# Autodesk Inventor assembly: 2026 Tiger Burn Head
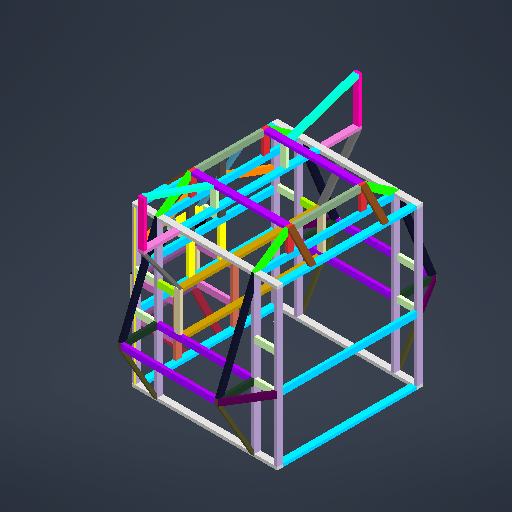
[picture p0: Inventor's stored thumbnail of the model, 512x512]
Saved by Autodesk Inventor 2027 (Build 310192000, 192)
## iProperties
Created: 2026-05-26
Part Number: 2026 Tiger Burn Head
Document SubType Name: Assembly
Designer: lucas
Author: lucas
## Documents named in this file (78)
- C:\Users\lucas\OneDrive\Documents\Inventor\Tiger Burn Head Frame 2026\2026 Tiger Burn Head.iam
- C:\Users\lucas\OneDrive\Documents\Inventor\Tiger Burn Head Frame 2026\2x4x96.ipt
- C:\Users\lucas\OneDrive\Documents\Inventor\Tiger Burn Head Frame 2026\2x4x88.ipt
- C:\Users\lucas\OneDrive\Documents\Inventor\Tiger Burn Head Frame 2026\2x4x101.ipt
- C:\Users\lucas\OneDrive\Documents\Inventor\Tiger Burn Head Frame 2026\2x4x24.ipt
- C:\Users\lucas\OneDrive\Documents\Inventor\Tiger Burn Head Frame 2026\2x4x26.ipt
- C:\Users\lucas\OneDrive\Documents\Inventor\Tiger Burn Head Frame 2026\2x4x39.ipt
- C:\Users\lucas\OneDrive\Documents\Inventor\Tiger Burn Head Frame 2026\2x4x38.ipt
- C:\Users\lucas\OneDrive\Documents\Inventor\Tiger Burn Head Frame 2026\Bottom jaw diagonals 2.ipt
- C:\Users\lucas\OneDrive\Documents\Inventor\Tiger Burn Head Frame 2026\Bottom jaw diagonals 2_MIR.ipt
- C:\Users\lucas\OneDrive\Documents\Inventor\Tiger Burn Head Frame 2026\2x4x24(with a cut).ipt
- C:\Users\lucas\OneDrive\Documents\Inventor\Tiger Burn Head Frame 2026\2x4x(24x43).ipt
- C:\Users\lucas\OneDrive\Documents\Inventor\Tiger Burn Head Frame 2026\Upper side diagonal.ipt
- C:\Users\lucas\OneDrive\Documents\Inventor\Tiger Burn Head Frame 2026\2x4x101_MIR.ipt
- C:\Users\lucas\OneDrive\Documents\Inventor\Tiger Burn Head Frame 2026\2x4x24(with a cut)_MIR.ipt
- C:\Users\lucas\OneDrive\Documents\Inventor\Tiger Burn Head Frame 2026\2x4x(24x43)_MIR.ipt
- C:\Users\lucas\OneDrive\Documents\Inventor\Tiger Burn Head Frame 2026\Upper side diagonal_MIR.ipt
- C:\Users\lucas\OneDrive\Documents\Inventor\Tiger Burn Head Frame 2026\2x4x101_MIR1.ipt
- C:\Users\lucas\OneDrive\Documents\Inventor\Tiger Burn Head Frame 2026\2x4x24(with a cut)_MIR1.ipt
- C:\Users\lucas\OneDrive\Documents\Inventor\Tiger Burn Head Frame 2026\2x4x(24x43)_MIR1.ipt
- C:\Users\lucas\OneDrive\Documents\Inventor\Tiger Burn Head Frame 2026\Upper side diagonal_MIR1.ipt
- C:\Users\lucas\OneDrive\Documents\Inventor\Tiger Burn Head Frame 2026\2x4x101_MIR_MIR.ipt
- C:\Users\lucas\OneDrive\Documents\Inventor\Tiger Burn Head Frame 2026\2x4x24(with a cut)_MIR_MIR.ipt
- C:\Users\lucas\OneDrive\Documents\Inventor\Tiger Burn Head Frame 2026\2x4x(24x43)_MIR_MIR.ipt
- C:\Users\lucas\OneDrive\Documents\Inventor\Tiger Burn Head Frame 2026\Upper side diagonal_MIR_MIR.ipt
- C:\Users\lucas\OneDrive\Documents\Inventor\Tiger Burn Head Frame 2026\Side piece.ipt
- C:\Users\lucas\OneDrive\Documents\Inventor\Tiger Burn Head Frame 2026\Side piece_MIR.ipt
- C:\Users\lucas\OneDrive\Documents\Inventor\Tiger Burn Head Frame 2026\2x4x15.ipt
- C:\Users\lucas\OneDrive\Documents\Inventor\Tiger Burn Head Frame 2026\2x4x44.ipt
- C:\Users\lucas\OneDrive\Documents\Inventor\Tiger Burn Head Frame 2026\Top of head diagonals.ipt
- C:\Users\lucas\OneDrive\Documents\Inventor\Tiger Burn Head Frame 2026\Top of head diagonals_MIR2.ipt
- C:\Users\lucas\OneDrive\Documents\Inventor\Tiger Burn Head Frame 2026\2x4x88_MIR.ipt
- C:\Users\lucas\OneDrive\Documents\Inventor\Tiger Burn Head Frame 2026\2x4x15_MIR1.ipt
- C:\Users\lucas\OneDrive\Documents\Inventor\Tiger Burn Head Frame 2026\2x4x44_MIR1.ipt
- C:\Users\lucas\OneDrive\Documents\Inventor\Tiger Burn Head Frame 2026\Top of head diagonals_MIR3.ipt
- C:\Users\lucas\OneDrive\Documents\Inventor\Tiger Burn Head Frame 2026\Top of head diagonals_MIR2_MIR.ipt
- C:\Users\lucas\OneDrive\Documents\Inventor\Tiger Burn Head Frame 2026\Side piece_MIR1.ipt
- C:\Users\lucas\OneDrive\Documents\Inventor\Tiger Burn Head Frame 2026\2x4x13.ipt
- C:\Users\lucas\OneDrive\Documents\Inventor\Tiger Burn Head Frame 2026\2x4x13_MIR.ipt
- C:\Users\lucas\OneDrive\Documents\Inventor\Tiger Burn Head Frame 2026\2x4x13_MIR1.ipt
- C:\Users\lucas\OneDrive\Documents\Inventor\Tiger Burn Head Frame 2026\2x4x13_MIR_MIR.ipt
- C:\Users\lucas\OneDrive\Documents\Inventor\Tiger Burn Head Frame 2026\2x4x88_MIR1.ipt
- C:\Users\lucas\OneDrive\Documents\Inventor\Tiger Burn Head Frame 2026\SideConnectors.ipt
- C:\Users\lucas\OneDrive\Documents\Inventor\Tiger Burn Head Frame 2026\SideConnectors_MIR.ipt
- C:\Users\lucas\OneDrive\Documents\Inventor\Tiger Burn Head Frame 2026\SideConnectors_MIR1.ipt
- C:\Users\lucas\OneDrive\Documents\Inventor\Tiger Burn Head Frame 2026\SideConnectors_MIR_MIR.ipt
- C:\Users\lucas\OneDrive\Documents\Inventor\Tiger Burn Head Frame 2026\Side piece_MIR2.ipt
- C:\Users\lucas\OneDrive\Documents\Inventor\Tiger Burn Head Frame 2026\Top Diagonals.ipt
- C:\Users\lucas\OneDrive\Documents\Inventor\Tiger Burn Head Frame 2026\Top Diagonals_MIR.ipt
- C:\Users\lucas\OneDrive\Documents\Inventor\Tiger Burn Head Frame 2026\Top Diagonals_MIR1.ipt
- C:\Users\lucas\OneDrive\Documents\Inventor\Tiger Burn Head Frame 2026\Top Diagonals_MIR_MIR.ipt
- C:\Users\lucas\OneDrive\Documents\Inventor\Tiger Burn Head Frame 2026\2x4x20.ipt
- C:\Users\lucas\OneDrive\Documents\Inventor\Tiger Burn Head Frame 2026\2x4x20_MIR.ipt
- C:\Users\lucas\OneDrive\Documents\Inventor\Tiger Burn Head Frame 2026\2x4x13_MIR2.ipt
- C:\Users\lucas\OneDrive\Documents\Inventor\Tiger Burn Head Frame 2026\Eyelids.ipt
- C:\Users\lucas\OneDrive\Documents\Inventor\Tiger Burn Head Frame 2026\Eyelids_MIR.ipt
- C:\Users\lucas\OneDrive\Documents\Inventor\Tiger Burn Head Frame 2026\UpperNoseDiagonalsv2.ipt
- C:\Users\lucas\OneDrive\Documents\Inventor\Tiger Burn Head Frame 2026\UpperNoseDiagonalsv2_MIR.ipt
- C:\Users\lucas\OneDrive\Documents\Inventor\Tiger Burn Head Frame 2026\Rename.ipt
- C:\Users\lucas\OneDrive\Documents\Inventor\Tiger Burn Head Frame 2026\Rename_MIR.ipt
- C:\Users\lucas\OneDrive\Documents\Inventor\Tiger Burn Head Frame 2026\Renamev2.ipt
- Eyelidpt2.ipt
- C:\Users\lucas\OneDrive\Documents\Inventor\Tiger Burn Head Frame 2026\Renamev2_MIR.ipt
- C:\Users\lucas\OneDrive\Documents\Inventor\Tiger Burn Head Frame 2026\LowerEarDiagonals.ipt
- C:\Users\lucas\OneDrive\Documents\Inventor\Tiger Burn Head Frame 2026\2x4x24_MIR1.ipt
- C:\Users\lucas\OneDrive\Documents\Inventor\Tiger Burn Head Frame 2026\2x4x26_MIR.ipt
- C:\Users\lucas\OneDrive\Documents\Inventor\Tiger Burn Head Frame 2026\LowerEarDiagonals_MIR.ipt
- C:\Users\lucas\OneDrive\Documents\Inventor\Tiger Burn Head Frame 2026\2x4x30.ipt
- C:\Users\lucas\OneDrive\Documents\Inventor\Tiger Burn Head Frame 2026\2x4x30_MIR.ipt
- C:\Users\lucas\OneDrive\Documents\Inventor\Tiger Burn Head Frame 2026\UpperEarDiagonalv2.ipt
- C:\Users\lucas\OneDrive\Documents\Inventor\Tiger Burn Head Frame 2026\UpperEarDiagonalv2_MIR.ipt
- C:\Users\lucas\OneDrive\Documents\Inventor\Tiger Burn Head Frame 2026\2x4x90.ipt
- C:\Users\lucas\OneDrive\Documents\Inventor\Tiger Burn Head Frame 2026\2x4x(Rename).ipt
- C:\Users\lucas\OneDrive\Documents\Inventor\Tiger Burn Head Frame 2026\2x4x13_MIR3.ipt
- C:\Users\lucas\OneDrive\Documents\Inventor\Tiger Burn Head Frame 2026\2x4x(Rename)_MIR.ipt
- C:\Users\lucas\OneDrive\Documents\Inventor\Tiger Burn Head Frame 2026\2x4x13_MIR4.ipt
- C:\Users\lucas\OneDrive\Documents\Inventor\Tiger Burn Head Frame 2026\2x4x13_MIR3_MIR.ipt
- C:\Users\lucas\OneDrive\Documents\Inventor\Tiger Burn Head Frame 2026\2x4x13_MIR5.ipt
## Components (107 placed, 77 different names)
1. 2x4x96:1 — Mate:1, Flush:1, Flush:2, Mate:2, Flush:3, Flush:4, Mate:8, Flush:15, Flush:16, Mate:9, Flush:17, Flush:18, Mate:28, Flush:53, Mate:38
2. 2x4x88:1 — Mate:1, Flush:1, Flush:2
3. 2x4x88:2 — Mate:2, Flush:3, Flush:4, Mate:3, Flush:5, Flush:6, Mate:12, Flush:23, Mate:13, Flush:25, Flush:52
4. 2x4x96:2 — Mate:3, Flush:5, Flush:6, Mate:7, Flush:13, Flush:14, Mate:10, Flush:19, Flush:20, Mate:39
5. 2x4x101:1 — Mate:7, Flush:13, Flush:14, Flush:24, Flush:107, Flush:108, Mate:68, Flush:123, Flush:136, Flush:137, Mate:73
6. 2x4x96:3 — Flush:21, Flush:22, Flush:87, Mate:72, Flush:139, Mate:78, Flush:149
7. 2x4x88:3
8. 2x4x88:4 — Flush:116, Flush:130
9. 2x4x96:4 — Mate:11, Mate:37
10. 2x4x101:2 — Mate:10, Flush:19, Flush:20, Mate:11, Flush:21, Flush:22
11. 2x4x101:3 — Mate:8, Flush:15, Flush:16, Flush:26, Flush:28, Flush:54, Mate:80, Flush:157
12. 2x4x101:4 — Mate:9, Flush:17, Flush:18
13. 2x4x39:1 — Mate:12, Flush:23, Flush:24, Mate:14
14. 2x4x39:2 — Mate:13, Flush:25, Flush:26, Flush:27, Flush:47
15. 2x4x88:5 — Mate:14, Flush:27, Flush:28, Mate:24, Flush:48, Mate:27, Flush:57, Mate:67, Flush:122
16. 2x4x24:1 — Mate:21, Flush:41, Flush:42
17. 2x4x24:2 — Mate:23, Flush:45, Flush:46, Mate:24, Flush:48
18. 2x4x24:3 — Mate:22, Flush:43, Flush:44
19. 2x4x24:4 — Mate:20, Flush:39, Flush:40
20. 2x4x26:2 — Mate:17, Flush:33, Flush:34, Mate:19, Flush:37, Flush:38, Mate:21, Flush:41, Flush:42, Mate:23, Flush:45, Flush:46, Flush:47, Flush:49, Flush:50
21. 2x4x38:2 — Mate:17, Flush:33, Flush:34, Mate:18, Flush:35, Flush:36, Mate:26
22. 2x4x26:3 — Mate:18, Flush:35, Flush:36, Mate:20, Flush:39, Flush:40, Mate:22, Flush:43, Flush:44, Flush:131, Flush:132
23. 2x4x38:3 — Mate:19, Flush:37, Flush:38, Mate:25
24. Bottom jaw diagonals 2:1 — Flush:49, Flush:50, Flush:52
25. Bottom jaw diagonals 2_MIR:1
26. 2x4x101:5 — Mate:28, Flush:53, Flush:54, Flush:56, Mate:30, Flush:95, Flush:105, Flush:106
27. 2x4x24(with a cut):1 — Flush:56, Mate:30, Flush:57, Flush:58, Flush:59, Flush:60, Flush:61, Flush:62
28. 2x4x(24x45) — Flush:58, Flush:59, Flush:72, Flush:73
29. Upper side diagonal:1 — Flush:60, Flush:61, Flush:62
30. 2x4x101_MIR:1 — Mate:31, Flush:63, Mate:53, Flush:88, Flush:94
31. 2x4x24(with a cut)_MIR:1 — Mate:31, Flush:63, Mate:32, Mate:33, Mate:34, Mate:35, Mate:36, Flush:76, Flush:109
32. 2x4x(24x43)_MIR:1 — Mate:32, Mate:33, Flush:75
33. Upper side diagonal_MIR:1 — Mate:34, Mate:35, Mate:36
34. 2x4x101_MIR1:1 — Mate:40, Flush:64, Mate:64, Flush:103
35. 2x4x24(with a cut)_MIR1:1 — Mate:40, Flush:64, Mate:41, Mate:42, Mate:43, Mate:44, Mate:45, Flush:74, Flush:104
36. 2x4x(24x43)_MIR1:1 — Mate:41, Mate:42
37. Upper side diagonal_MIR1:1 — Mate:43, Mate:44, Mate:45
38. 2x4x101_MIR_MIR:1 — Flush:65, Mate:46
39. 2x4x24(with a cut)_MIR_MIR:1 — Flush:65, Mate:46, Flush:66, Flush:67, Flush:68, Flush:69, Flush:70
40. 2x4x(24x43)_MIR_MIR:1 — Flush:66, Flush:67, Flush:71
41. Upper side diagonal_MIR_MIR:1 — Flush:68, Flush:69, Flush:70
42. 2x4x62 — Flush:71, Flush:72, Flush:73, Flush:74
43. Side piece_MIR:1 — Flush:75, Flush:76
44. 2x4x88:6 — Mate:53, Flush:87, Flush:88, Mate:55, Flush:93, Mate:56, Flush:96, Mate:57, Flush:97
45. 2x4x15:3 — Mate:55, Flush:93, Flush:94, Mate:66, Flush:114, Flush:115
46. 2x4x15:4 — Mate:56, Flush:95, Flush:96, Mate:58, Flush:161
47. 2x4x44:2
48. Top of head diagonals:2 — Mate:57, Flush:97, Mate:58
49. Top of head diagonals_MIR2:1
50. 2x4x88_MIR:1 — Flush:98, Mate:59, Flush:99, Mate:60, Flush:102, Mate:63, Flush:113
51. 2x4x15_MIR1:1 — Flush:98, Mate:59, Flush:100, Flush:101, Mate:61, Flush:110, Flush:111, Flush:112, Flush:113
52. 2x4x15_MIR1:2 — Flush:99, Mate:60, Mate:62
53. 2x4x44_MIR1:1 — Flush:100, Flush:101, Mate:61
54. Top of head diagonals_MIR3:1 — Mate:62, Flush:102, Mate:63
55. Top of head diagonals_MIR2_MIR:1 — Flush:112
56. Side piece:2 — Mate:64, Flush:103, Flush:104, Mate:79, Flush:156
57. Side piece_MIR1:1 — Mate:74, Flush:140
58. 2x4x13:1 — Flush:105, Flush:106
59. 2x4x13_MIR:1
60. 2x4x13_MIR1:1
61. 2x4x13_MIR_MIR:1
62. 2x4x88_MIR1:1 — Mate:65
63. SideConnectors:1 — Flush:107, Flush:108, Flush:109
64. SideConnectors_MIR:1
65. SideConnectors_MIR1:1
66. SideConnectors_MIR_MIR:1
67. Side piece:3 — Flush:110, Flush:111, Mate:66, Flush:152
68. Side piece_MIR2:1
69. Top Diagonals:1 — Flush:114, Flush:115, Flush:116
70. Top Diagonals_MIR:1
71. Top Diagonals_MIR1:1
72. Top Diagonals_MIR_MIR:1
73. 2x4x20:2 — Mate:67, Flush:122, Mate:69, Flush:124
74. 2x4x20_MIR:1
75. 2x4x88:7 — Mate:68, Flush:123, Mate:69, Flush:125, Mate:70, Flush:134, Flush:135, Flush:158
76. 2x4x13:2 — Flush:124, Flush:125, Mate:70, Flush:126, Mate:71, Flush:127, Flush:128, Flush:129, Flush:133
77. 2x4x13_MIR2:1
78. 2x4x20:3 — Flush:126, Mate:71, Flush:127
79. Eyelids:1 — Flush:128, Flush:129, Flush:130
80. Eyelids_MIR:1
81. UpperNoseDiagonalsv2:1 — Flush:131, Flush:132, Flush:133
82. UpperNoseDiagonalsv2_MIR:1
83. 2x4x34:1 — Flush:134, Flush:135, Flush:138
84. 2x4x34_MIR:1
85. Eyelidpt2:1 — Flush:136, Flush:137, Flush:138
86. Eyelidpt2_MIR:1
87. 2x4x24:5 — Mate:72, Flush:139, Mate:73, Flush:141, Flush:144, Flush:146, Flush:147, Flush:148
88. 2x4x26:4 — Mate:74, Flush:140, Flush:141, Flush:142, Flush:143, Flush:153, Flush:154
89. LowerEarDiagonals:1 — Flush:142, Flush:143, Flush:144
90. 2x4x24_MIR1:1 — Flush:145, Mate:75
91. 2x4x26_MIR:1 — Flush:145, Mate:76, Mate:77, Flush:155, Flush:159, Flush:160
92. LowerEarDiagonals_MIR:1 — Mate:75, Mate:76, Mate:77
93. 2x4x30:1 — Flush:146, Flush:147, Flush:150, Flush:151
94. 2x4x88:8 — Mate:78, Flush:148, Flush:149, Mate:81
95. 2x4x30_MIR:1
96. UpperEarDiagonalv2:1 — Flush:150, Flush:151, Flush:152
97. UpperEarDiagonalv2_MIR:1
98. 2x4x92:1 — Flush:153, Flush:154
99. 2x4x92:2 — Mate:79, Flush:155, Flush:156
100. 2x4x13:3 — Mate:80, Flush:157, Flush:158
101. 2x4x11:1 — Flush:159, Flush:160
102. 2x4x13_MIR3:1
103. 2x4x(Rename)_MIR:1
104. 2x4x13_MIR4:1
105. 2x4x13_MIR3_MIR:1
106. 2x4x13:4 — Mate:81, Flush:161
107. 2x4x13_MIR5:1
## Relationships (210: Flush 138, Mate 72)
- Mate:1: 2x4x96:1 ↔ 2x4x88:1
- Flush:1: 2x4x96:1 ↔ 2x4x88:1
- Flush:2: 2x4x96:1 ↔ 2x4x88:1
- Mate:2: 2x4x96:1 ↔ 2x4x88:2
- Flush:3: 2x4x96:1 ↔ 2x4x88:2
- Flush:4: 2x4x96:1 ↔ 2x4x88:2
- Mate:3: 2x4x88:2 ↔ 2x4x96:2
- Flush:5: 2x4x88:2 ↔ 2x4x96:2
- Flush:6: 2x4x88:2 ↔ 2x4x96:2
- [Mate]: 2x4x96:3 ↔ 2x4x88:3
- [Flush]: 2x4x96:3 ↔ 2x4x88:3
- [Flush]: 2x4x96:3 ↔ 2x4x88:3
- [Mate]: 2x4x96:3 ↔ 2x4x88:4
- [Flush]: 2x4x96:3 ↔ 2x4x88:4
- [Flush]: 2x4x96:3 ↔ 2x4x88:4
- [Mate]: 2x4x88:4 ↔ 2x4x96:4
- [Flush]: 2x4x88:4 ↔ 2x4x96:4
- [Flush]: 2x4x88:4 ↔ 2x4x96:4
- Mate:7: 2x4x96:2 ↔ 2x4x101:1
- Flush:13: 2x4x96:2 ↔ 2x4x101:1
- Flush:14: 2x4x96:2 ↔ 2x4x101:1
- Mate:8: 2x4x96:1 ↔ 2x4x101:3
- Flush:15: 2x4x96:1 ↔ 2x4x101:3
- Flush:16: 2x4x96:1 ↔ 2x4x101:3
- Mate:9: 2x4x96:1 ↔ 2x4x101:4
- Flush:17: 2x4x96:1 ↔ 2x4x101:4
- Flush:18: 2x4x96:1 ↔ 2x4x101:4
- Mate:10: 2x4x96:2 ↔ 2x4x101:2
- Flush:19: 2x4x96:2 ↔ 2x4x101:2
- Flush:20: 2x4x96:2 ↔ 2x4x101:2
- Mate:11: 2x4x96:4 ↔ 2x4x101:2
- Flush:21: 2x4x96:3 ↔ 2x4x101:2
- Flush:22: 2x4x96:3 ↔ 2x4x101:2
- Mate:12: 2x4x88:2 ↔ 2x4x39:1
- Flush:23: 2x4x88:2 ↔ 2x4x39:1
- Flush:24 (685.8 mm): 2x4x101:1 ↔ 2x4x39:1
- Mate:13: 2x4x88:2 ↔ 2x4x39:2
- Flush:25: 2x4x88:2 ↔ 2x4x39:2
- Flush:26 (685.8 mm): 2x4x101:3 ↔ 2x4x39:2
- Mate:14: 2x4x39:1 ↔ 2x4x88:5
- Flush:27: 2x4x39:2 ↔ 2x4x88:5
- Flush:28 (101.6 mm): 2x4x101:3 ↔ 2x4x88:5
- Mate:17: 2x4x26:2 ↔ 2x4x38:2
- Flush:33: 2x4x26:2 ↔ 2x4x38:2
- Flush:34: 2x4x26:2 ↔ 2x4x38:2
- Mate:18: 2x4x38:2 ↔ 2x4x26:3
- Flush:35: 2x4x38:2 ↔ 2x4x26:3
- Flush:36: 2x4x38:2 ↔ 2x4x26:3
- Mate:19: 2x4x26:2 ↔ 2x4x38:3
- Flush:37: 2x4x26:2 ↔ 2x4x38:3
- Flush:38: 2x4x26:2 ↔ 2x4x38:3
- Mate:20: 2x4x24:4 ↔ 2x4x26:3
- Flush:39: 2x4x24:4 ↔ 2x4x26:3
- Flush:40: 2x4x24:4 ↔ 2x4x26:3
- Mate:21: 2x4x24:1 ↔ 2x4x26:2
- Flush:41: 2x4x24:1 ↔ 2x4x26:2
- Flush:42: 2x4x24:1 ↔ 2x4x26:2
- Mate:22: 2x4x24:3 ↔ 2x4x26:3
- Flush:43: 2x4x24:3 ↔ 2x4x26:3
- Flush:44: 2x4x24:3 ↔ 2x4x26:3
- Mate:23: 2x4x24:2 ↔ 2x4x26:2
- Flush:45: 2x4x24:2 ↔ 2x4x26:2
- Flush:46: 2x4x24:2 ↔ 2x4x26:2
- Mate:24: 2x4x88:5 ↔ 2x4x24:2
- Flush:47: 2x4x39:2 ↔ 2x4x26:2
- Flush:48 (203.2 mm): 2x4x88:5 ↔ 2x4x24:2
- Flush:49: 2x4x26:2 ↔ Bottom jaw diagonals 2:1
- Flush:50: 2x4x26:2 ↔ Bottom jaw diagonals 2:1
- Flush:52: 2x4x88:2 ↔ Bottom jaw diagonals 2:1
- Mate:25: 2x4x38:3
- Mate:26: 2x4x38:2
- Mate:27: 2x4x88:5
- Mate:28: 2x4x96:1 ↔ 2x4x101:5
- Flush:53: 2x4x96:1 ↔ 2x4x101:5
- Flush:54 (-381 mm): 2x4x101:3 ↔ 2x4x101:5
- Flush:56: 2x4x101:5 ↔ 2x4x24(with a cut):1
- Mate:30: 2x4x101:5 ↔ 2x4x24(with a cut):1
- Flush:57: 2x4x88:5 ↔ 2x4x24(with a cut):1
- Flush:58: 2x4x24(with a cut):1 ↔ 2x4x(24x45)
- Flush:59: 2x4x24(with a cut):1 ↔ 2x4x(24x45)
- Flush:60: 2x4x24(with a cut):1 ↔ Upper side diagonal:1
- Flush:61: 2x4x24(with a cut):1 ↔ Upper side diagonal:1
- Flush:62: 2x4x24(with a cut):1 ↔ Upper side diagonal:1
- Mate:31: 2x4x101_MIR:1 ↔ 2x4x24(with a cut)_MIR:1
- Flush:63: 2x4x101_MIR:1 ↔ 2x4x24(with a cut)_MIR:1
- Mate:32: 2x4x24(with a cut)_MIR:1 ↔ 2x4x(24x43)_MIR:1
- Mate:33: 2x4x24(with a cut)_MIR:1 ↔ 2x4x(24x43)_MIR:1
- Mate:34: 2x4x24(with a cut)_MIR:1 ↔ Upper side diagonal_MIR:1
- Mate:35: 2x4x24(with a cut)_MIR:1 ↔ Upper side diagonal_MIR:1
- Mate:36: 2x4x24(with a cut)_MIR:1 ↔ Upper side diagonal_MIR:1
- Mate:37: 2x4x96:4
- Mate:38: 2x4x96:1
- Mate:39: 2x4x96:2
- Mate:40: 2x4x101_MIR1:1 ↔ 2x4x24(with a cut)_MIR1:1
- Flush:64: 2x4x101_MIR1:1 ↔ 2x4x24(with a cut)_MIR1:1
- Mate:41: 2x4x24(with a cut)_MIR1:1 ↔ 2x4x(24x43)_MIR1:1
- Mate:42: 2x4x24(with a cut)_MIR1:1 ↔ 2x4x(24x43)_MIR1:1
- Mate:43: 2x4x24(with a cut)_MIR1:1 ↔ Upper side diagonal_MIR1:1
- Mate:44: 2x4x24(with a cut)_MIR1:1 ↔ Upper side diagonal_MIR1:1
- Mate:45: 2x4x24(with a cut)_MIR1:1 ↔ Upper side diagonal_MIR1:1
- Flush:65: 2x4x101_MIR_MIR:1 ↔ 2x4x24(with a cut)_MIR_MIR:1
- Mate:46: 2x4x101_MIR_MIR:1 ↔ 2x4x24(with a cut)_MIR_MIR:1
- Flush:66: 2x4x24(with a cut)_MIR_MIR:1 ↔ 2x4x(24x43)_MIR_MIR:1
- Flush:67: 2x4x24(with a cut)_MIR_MIR:1 ↔ 2x4x(24x43)_MIR_MIR:1
- Flush:68: 2x4x24(with a cut)_MIR_MIR:1 ↔ Upper side diagonal_MIR_MIR:1
- Flush:69: 2x4x24(with a cut)_MIR_MIR:1 ↔ Upper side diagonal_MIR_MIR:1
- Flush:70: 2x4x24(with a cut)_MIR_MIR:1 ↔ Upper side diagonal_MIR_MIR:1
- Flush:71: 2x4x(24x43)_MIR_MIR:1 ↔ 2x4x62
- Flush:72: 2x4x(24x45) ↔ 2x4x62
- Flush:73: 2x4x(24x45) ↔ 2x4x62
- Flush:74: 2x4x24(with a cut)_MIR1:1 ↔ 2x4x62
- Flush:75: 2x4x(24x43)_MIR:1 ↔ Side piece_MIR:1
- Flush:76: 2x4x24(with a cut)_MIR:1 ↔ Side piece_MIR:1
- Mate:53: 2x4x101_MIR:1 ↔ 2x4x88:6
- Flush:87: 2x4x96:3 ↔ 2x4x88:6
- Flush:88: 2x4x101_MIR:1 ↔ 2x4x88:6
- [Mate]: 2x4x15:3 ↔ 2x4x44:2
- [Flush]: 2x4x15:3 ↔ 2x4x44:2
- [Flush]: 2x4x15:3 ↔ 2x4x44:2
- Mate:55: 2x4x88:6 ↔ 2x4x15:3
- Flush:93: 2x4x88:6 ↔ 2x4x15:3
- Flush:94 (-558.8 mm): 2x4x101_MIR:1 ↔ 2x4x15:3
- Mate:56: 2x4x88:6 ↔ 2x4x15:4
- Flush:95 (558.8 mm): 2x4x101:5 ↔ 2x4x15:4
- Flush:96: 2x4x88:6 ↔ 2x4x15:4
- Mate:57: 2x4x88:6 ↔ Top of head diagonals:2
- Flush:97: 2x4x88:6 ↔ Top of head diagonals:2
- Mate:58: 2x4x15:4 ↔ Top of head diagonals:2
- Flush:98: 2x4x88_MIR:1 ↔ 2x4x15_MIR1:1
- Mate:59: 2x4x88_MIR:1 ↔ 2x4x15_MIR1:1
- Flush:99: 2x4x88_MIR:1 ↔ 2x4x15_MIR1:2
- Mate:60: 2x4x88_MIR:1 ↔ 2x4x15_MIR1:2
- Flush:100: 2x4x15_MIR1:1 ↔ 2x4x44_MIR1:1
- Flush:101: 2x4x15_MIR1:1 ↔ 2x4x44_MIR1:1
- Mate:61: 2x4x15_MIR1:1 ↔ 2x4x44_MIR1:1
- Mate:62: 2x4x15_MIR1:2 ↔ Top of head diagonals_MIR3:1
- Flush:102: 2x4x88_MIR:1 ↔ Top of head diagonals_MIR3:1
- Mate:63: 2x4x88_MIR:1 ↔ Top of head diagonals_MIR3:1
- Mate:64: 2x4x101_MIR1:1 ↔ Side piece:2
- Flush:103: 2x4x101_MIR1:1 ↔ Side piece:2
- Flush:104: 2x4x24(with a cut)_MIR1:1 ↔ Side piece:2
- Flush:105: 2x4x101:5 ↔ 2x4x13:1
- Flush:106: 2x4x101:5 ↔ 2x4x13:1
- Mate:65: 2x4x88_MIR1:1
- Flush:107: 2x4x101:1 ↔ SideConnectors:1
- Flush:108: 2x4x101:1 ↔ SideConnectors:1
- Flush:109: 2x4x24(with a cut)_MIR:1 ↔ SideConnectors:1
- Flush:110: 2x4x15_MIR1:1 ↔ Side piece:3
- Flush:111: 2x4x15_MIR1:1 ↔ Side piece:3
- Flush:112: 2x4x15_MIR1:1 ↔ Top of head diagonals_MIR2_MIR:1
- Flush:113: 2x4x88_MIR:1 ↔ 2x4x15_MIR1:1
- Mate:66: 2x4x15:3 ↔ Side piece:3
- Flush:114: 2x4x15:3 ↔ Top Diagonals:1
- Flush:115: 2x4x15:3 ↔ Top Diagonals:1
- Flush:116: 2x4x88:4 ↔ Top Diagonals:1
- Mate:67: 2x4x88:5 ↔ 2x4x20:2
- Flush:122: 2x4x88:5 ↔ 2x4x20:2
- Mate:68: 2x4x101:1 ↔ 2x4x88:7
- Flush:123: 2x4x101:1 ↔ 2x4x88:7
- Mate:69: 2x4x20:2 ↔ 2x4x88:7
- Flush:124: 2x4x20:2 ↔ 2x4x13:2
- Flush:125: 2x4x88:7 ↔ 2x4x13:2
- Mate:70: 2x4x88:7 ↔ 2x4x13:2
- Flush:126: 2x4x13:2 ↔ 2x4x20:3
- Mate:71: 2x4x13:2 ↔ 2x4x20:3
- Flush:127: 2x4x13:2 ↔ 2x4x20:3
- Flush:128: 2x4x13:2 ↔ Eyelids:1
- Flush:129: 2x4x13:2 ↔ Eyelids:1
- Flush:130: 2x4x88:4 ↔ Eyelids:1
- Flush:131: 2x4x26:3 ↔ UpperNoseDiagonalsv2:1
- Flush:132: 2x4x26:3 ↔ UpperNoseDiagonalsv2:1
- Flush:133: 2x4x13:2 ↔ UpperNoseDiagonalsv2:1
- Flush:134: 2x4x88:7 ↔ 2x4x34:1
- Flush:135: 2x4x88:7 ↔ 2x4x34:1
- Flush:136: 2x4x101:1 ↔ Eyelidpt2:1
- Flush:137: 2x4x101:1 ↔ Eyelidpt2:1
- Flush:138: 2x4x34:1 ↔ Eyelidpt2:1
- Mate:72: 2x4x96:3 ↔ 2x4x24:5
- Flush:139: 2x4x96:3 ↔ 2x4x24:5
- Mate:73 (660.4 mm): 2x4x101:1 ↔ 2x4x24:5
- Mate:74: Side piece_MIR1:1 ↔ 2x4x26:4
- Flush:140: Side piece_MIR1:1 ↔ 2x4x26:4
- Flush:141: 2x4x24:5 ↔ 2x4x26:4
- Flush:142: 2x4x26:4 ↔ LowerEarDiagonals:1
- Flush:143: 2x4x26:4 ↔ LowerEarDiagonals:1
- Flush:144: 2x4x24:5 ↔ LowerEarDiagonals:1
- Flush:145: 2x4x24_MIR1:1 ↔ 2x4x26_MIR:1
- Mate:75: 2x4x24_MIR1:1 ↔ LowerEarDiagonals_MIR:1
- Mate:76: 2x4x26_MIR:1 ↔ LowerEarDiagonals_MIR:1
- Mate:77: 2x4x26_MIR:1 ↔ LowerEarDiagonals_MIR:1
- Flush:146: 2x4x24:5 ↔ 2x4x30:1
- Flush:147: 2x4x24:5 ↔ 2x4x30:1
- Mate:78: 2x4x96:3 ↔ 2x4x88:8
- Flush:148: 2x4x24:5 ↔ 2x4x88:8
- Flush:149: 2x4x96:3 ↔ 2x4x88:8
- Flush:150: 2x4x30:1 ↔ UpperEarDiagonalv2:1
- Flush:151: 2x4x30:1 ↔ UpperEarDiagonalv2:1
- Flush:152: Side piece:3 ↔ UpperEarDiagonalv2:1
- Flush:153: 2x4x26:4 ↔ 2x4x92:1
- Flush:154: 2x4x26:4 ↔ 2x4x92:1
- Mate:79: Side piece:2 ↔ 2x4x92:2
- Flush:155: 2x4x26_MIR:1 ↔ 2x4x92:2
- Flush:156: Side piece:2 ↔ 2x4x92:2
- Mate:80: 2x4x101:3 ↔ 2x4x13:3
- Flush:157: 2x4x101:3 ↔ 2x4x13:3
- Flush:158: 2x4x88:7 ↔ 2x4x13:3
- Flush:159: 2x4x26_MIR:1 ↔ 2x4x11:1
- Flush:160: 2x4x26_MIR:1 ↔ 2x4x11:1
- Mate:81: 2x4x88:8 ↔ 2x4x13:4
- Flush:161: 2x4x15:4 ↔ 2x4x13:4
## Named parameters: d9_d4 = 0 mm, d10_d5 = 0 mm, d11_d6 = 0 mm, d12_d7 = 0 mm, d13_d8 = 0 mm, d14_d0 = 0 mm, d15_d1 = 0 mm, d16_d2 = 0 mm, d17_d3 = 0 mm, d224_d211 = 0 mm, d225_d212 = 0 mm, d226_d213 = 0 mm
